# Autodesk Inventor assembly: FloatingBarChair
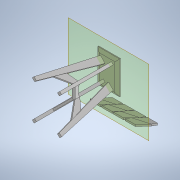
[picture p0: Inventor's stored thumbnail of the model, 180x180]
Saved by Autodesk Inventor 2022 (Build 260153000, 153)
## iProperties
Created: 2021-12-19
Part Number: FloatingBarChair
Document SubType Name: Assembly
Designer: dangl
Author: dangl
## Documents named in this file (8)
- C:\Users\dangl\Documents\WoodWork\FloatingBarChair\FloatingBarChair.iam
- C:\Users\dangl\Documents\WoodWork\FloatingBarChair\ChairTop.ipt
- C:\Users\dangl\Documents\WoodWork\FloatingBarChair\Leg.ipt
- C:\Users\dangl\Documents\WoodWork\FloatingBarChair\LegConnector.ipt
- C:\Users\dangl\Documents\WoodWork\FloatingBarChair\LegConnector_MIR.ipt
- C:\Users\dangl\Documents\WoodWork\FloatingBarChair\LegConnector_MIR1.ipt
- C:\Users\dangl\Documents\WoodWork\FloatingBarChair\LegConnector_MIR_MIR.ipt
- C:\Users\dangl\Documents\WoodWork\FloatingBarChair\LegConnectorBase.ipt
## Components (18 placed, 7 different names)
1. ChairTop:1 — Flush:1, Flush:2, Mate:5, Flush:4, Flush:5, Flush:6
2. Leg:1 — Flush:1, Flush:2, Mate:2, Mate:3, Mate:4, Mate:6, Mate:7, Flush:3
3. Leg:2 — Mate:3, Mate:4
4. Leg:3 — Mate:2, Mate:5
5. Leg:4 — Mate:6, Mate:7
6. LegConnector:1 — Flush:3, Flush:4
7. LegConnector_MIR:1
8. LegConnector_MIR1:1
9. LegConnector_MIR_MIR:1
10. LegConnectorBase:1 — Flush:5, Flush:6
11. LegConnector:2 — Mate:8, Flush:7, Mate:11, Mate:13
12. LegConnector:3 — Mate:8, Flush:7, Flush:9, Mate:11, Mate:12, Flush:12
13. LegConnector:4 — Mate:10, Flush:12, Mate:13, Mate:14, Mate:15, Flush:13, Flush:14, Flush:15, Flush:17, Flush:18
14. LegConnector:5 — Flush:9, Mate:10, Mate:15, Mate:16
15. LegConnector:6 — Flush:13, Flush:15, Flush:16, Mate:16, Mate:17, Mate:20
16. LegConnector:7 — Flush:14, Flush:16, Mate:18, Mate:19, Mate:21
17. LegConnector:8 — Flush:17, Mate:17, Mate:19, Mate:20
18. LegConnector:9 — Flush:18, Mate:18, Mate:21
## Relationships (34: Mate 19, Flush 15)
- Flush:1: ChairTop:1 ↔ Leg:1
- Flush:2: ChairTop:1 ↔ Leg:1
- Mate:2: Leg:1 ↔ Leg:3
- Mate:3: Leg:1 ↔ Leg:2
- Mate:4: Leg:1 ↔ Leg:2
- Mate:5: ChairTop:1 ↔ Leg:3
- Mate:6: Leg:1 ↔ Leg:4
- Mate:7: Leg:1 ↔ Leg:4
- Flush:3: Leg:1 ↔ LegConnector:1
- Flush:4: ChairTop:1 ↔ LegConnector:1
- Flush:5: ChairTop:1 ↔ LegConnectorBase:1
- Flush:6: ChairTop:1 ↔ LegConnectorBase:1
- Mate:8: LegConnector:2 ↔ LegConnector:3
- Flush:7: LegConnector:2 ↔ LegConnector:3
- Flush:9: LegConnector:3 ↔ LegConnector:5
- Mate:10: LegConnector:4 ↔ LegConnector:5
- Mate:11: LegConnector:2 ↔ LegConnector:3
- Mate:12: LegConnector:3
- Flush:12: LegConnector:3 ↔ LegConnector:4
- Mate:13: LegConnector:2 ↔ LegConnector:4
- Mate:14: LegConnector:4
- Mate:15: LegConnector:4 ↔ LegConnector:5
- Flush:13: LegConnector:4 ↔ LegConnector:6
- Flush:14: LegConnector:4 ↔ LegConnector:7
- Flush:15: LegConnector:4 ↔ LegConnector:6
- Flush:16: LegConnector:6 ↔ LegConnector:7
- Mate:16: LegConnector:5 ↔ LegConnector:6
- Flush:17: LegConnector:4 ↔ LegConnector:8
- Flush:18: LegConnector:4 ↔ LegConnector:9
- Mate:17: LegConnector:6 ↔ LegConnector:8
- Mate:18: LegConnector:7 ↔ LegConnector:9
- Mate:19: LegConnector:7 ↔ LegConnector:8
- Mate:20: LegConnector:6 ↔ LegConnector:8
- Mate:21: LegConnector:7 ↔ LegConnector:9
